# Autodesk Inventor assembly: Knee_MIR
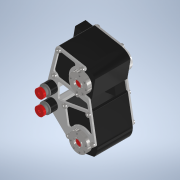
[picture p0: Inventor's stored thumbnail of the model, 180x180]
Saved by Autodesk Inventor 2020 (Build 240168000, 168)
## iProperties
Created: 2021-09-06
Part Number: Knee_MIR
Document SubType Name: Assembly
Designer: Masato Kubotera
Mass: 264.861 g
Surface Area: 473.637 cm^2
Volume: 130.531 cm^3
Density: 2.0291 g/cm^3
Author: Masato
## Documents named in this file (16)
- C:\Users\Masato\Desktop\OpenPlatform_ver3_0 - Ver4_1branch\LowerBody\Knee\Knee_MIR.iam
- C:\Users\Masato\Desktop\OpenPlatform_ver3_0 - Ver4_1branch\LowerBody\Knee\Knee_side_frame.ipt
- C:\Users\Masato\Desktop\OpenPlatform_ver3_0 - Ver4_1branch\Ready_Made\B3M11xx.ipt
- C:\Users\Masato\Desktop\OpenPlatform_ver3_0 - Ver4_1branch\Ready_Made\ClampHorn.ipt
- C:\Users\Masato\Desktop\OpenPlatform_ver3_0 - Ver4_1branch\Ready_Made\Screw\ClampHorn_Screw.ipt
- C:\Users\Masato\Desktop\OpenPlatform_ver3_0 - Ver4_1branch\Ready_Made\FreeHorn.ipt
- C:\Users\Masato\Desktop\OpenPlatform_ver3_0 - Ver4_1branch\Ready_Made\Screw\FreeHorn_Screw.ipt
- C:\Users\Masato\Desktop\OpenPlatform_ver3_0 - Ver4_1branch\Ready_Made\80F-0603.ipt
- C:\Users\Masato\Desktop\OpenPlatform_ver3_0 - Ver4_1branch\Ready_Made\Screw\M2_6-15.ipt
- C:\Users\Masato\Desktop\OpenPlatform_ver3_0 - Ver4_1branch\Ready_Made\Screw\M2_6-20.ipt
- C:\Users\Masato\Desktop\OpenPlatform_ver3_0 - Ver4_1branch\Ready_Made\UUW-0412-10BH.ipt
- C:\Users\Masato\Desktop\OpenPlatform_ver3_0 - Ver4_1branch\Ready_Made\CC-0612-15B.ipt
- C:\Users\Masato\Desktop\OpenPlatform_ver3_0 - Ver4_1branch\Ready_Made\CC-0612-50B.ipt
- C:\Users\Masato\Desktop\OpenPlatform_ver3_0 - Ver4_1branch\Ready_Made\SLSBF6-39_5-M4-N4.ipt
- C:\Users\Masato\Desktop\OpenPlatform_ver3_0 - Ver4_1branch\Ready_Made\DBTS4-11-6.ipt
- ClampHorn.ipt
## Components (50 placed, 14 different names)
1. Knee_side_frame:1 — フラッシュ:1, メイト:2, メイト:1, 挿入:6, 挿入:5, 挿入:8, 挿入:7, 挿入:3, 挿入:4, 挿入:1, 挿入:2, 挿入:9, 挿入:10, 挿入:12, 挿入:11, 挿入:13, 挿入:14, 挿入:15, 挿入:16, 角度:1, 挿入:33, 挿入:34, 挿入:37, 挿入:38
2. Knee_side_frame:2 — 挿入:22, 挿入:24, 挿入:21, 挿入:23, 挿入:20, 挿入:19, 挿入:18, 挿入:17, 挿入:26, 挿入:25, 挿入:28, 挿入:27, 挿入:31, 挿入:30, 挿入:32, 挿入:29, 挿入:35, 挿入:36, 挿入:39, 挿入:40
3. B3M11xx:1 — 挿入:20, 挿入:19, 挿入:3, 挿入:4, 挿入:18, 挿入:17, 挿入:1, 挿入:2, 挿入:61, 挿入:63, 挿入:59, 角度:3, 挿入:57
4. B3M11xx:2 — 挿入:6, 挿入:22, 挿入:24, 挿入:21, 挿入:23, 挿入:5, 挿入:8, 挿入:7, 挿入:62, 挿入:64, 挿入:60, 角度:4, 挿入:58
5. ClampHorn:1 — フラッシュ:2, 挿入:57, 角度:3
6. ClampHorn:2 — フラッシュ:3, 挿入:58, 角度:4
7. ClampHorn_Screw:1 — 挿入:59
8. ClampHorn_Screw:2 — 挿入:60
9. FreeHorn:1 — 挿入:61, フラッシュ:2
10. FreeHorn:2 — 挿入:62, フラッシュ:3
11. FreeHorn_Screw:1 — 挿入:63
12. FreeHorn_Screw:2 — 挿入:64
13. 80F-0603:1 — 挿入:49
14. 80F-0603:2 — 挿入:50
15. 80F-0603:3 — 挿入:51
16. 80F-0603:4 — 挿入:52
17. M2_6-15:1 — 挿入:9
18. M2_6-15:2 — 挿入:10
19. M2_6-15:3 — 挿入:11
20. M2_6-15:4 — 挿入:12
21. M2_6-15:5 — 挿入:13
22. M2_6-15:6 — 挿入:14
23. M2_6-15:7 — 挿入:15
24. M2_6-15:8 — 挿入:16
25. M2_6-20:1 — 挿入:25
26. M2_6-20:2 — 挿入:26
27. M2_6-20:3 — 挿入:27
28. M2_6-20:4 — 挿入:28
29. M2_6-20:5 — 挿入:29
30. M2_6-20:6 — 挿入:30
31. M2_6-20:7 — 挿入:31
32. M2_6-20:8 — 挿入:32
33. UUW-0412-10BH:1 — 挿入:53, 挿入:41, 挿入:37
34. UUW-0412-10BH:2 — 挿入:38, 挿入:54, 挿入:42
35. UUW-0412-10BH:3 — 挿入:55, 挿入:43, 挿入:39
36. UUW-0412-10BH:4 — 挿入:40, 挿入:56, 挿入:44
37. CC-0612-15B:1 — 挿入:45, 挿入:41
38. CC-0612-15B:2 — 挿入:46, 挿入:42
39. CC-0612-15B:3 — 挿入:47, 挿入:43
40. CC-0612-15B:4 — 挿入:48, 挿入:44
41. CC-0612-50B:1 — 挿入:49, 挿入:45
42. CC-0612-50B:2 — 挿入:50, 挿入:46
43. CC-0612-50B:3 — 挿入:51, 挿入:47
44. CC-0612-50B:4 — 挿入:52, 挿入:48
45. SLSBF6-39_5-M4-N4:1 — 角度:1, 挿入:33, 挿入:35, 角度:2
46. SLSBF6-39_5-M4-N4:2 — 挿入:36, 挿入:34, 角度:2
47. DBTS4-11-6:1 — 挿入:53
48. DBTS4-11-6:2 — 挿入:54
49. DBTS4-11-6:3 — 挿入:55
50. DBTS4-11-6:4 — 挿入:56
## Relationships (73: Insert 64, Angle 4, Flush 3, Mate 2)
- フラッシュ:1 [Flush]: Knee_side_frame:1
- メイト:2 [Mate] (19.75 mm): Knee_side_frame:1
- メイト:1 [Mate]: Knee_side_frame:1
- 挿入:6 [Insert]: Knee_side_frame:1 ↔ B3M11xx:2
- 挿入:22 [Insert]: Knee_side_frame:2 ↔ B3M11xx:2
- 挿入:24 [Insert]: Knee_side_frame:2 ↔ B3M11xx:2
- 挿入:21 [Insert]: Knee_side_frame:2 ↔ B3M11xx:2
- 挿入:23 [Insert]: Knee_side_frame:2 ↔ B3M11xx:2
- 挿入:5 [Insert]: Knee_side_frame:1 ↔ B3M11xx:2
- 挿入:8 [Insert]: Knee_side_frame:1 ↔ B3M11xx:2
- 挿入:7 [Insert]: Knee_side_frame:1 ↔ B3M11xx:2
- 挿入:20 [Insert]: Knee_side_frame:2 ↔ B3M11xx:1
- 挿入:19 [Insert]: Knee_side_frame:2 ↔ B3M11xx:1
- 挿入:3 [Insert]: Knee_side_frame:1 ↔ B3M11xx:1
- 挿入:4 [Insert]: Knee_side_frame:1 ↔ B3M11xx:1
- 挿入:18 [Insert]: Knee_side_frame:2 ↔ B3M11xx:1
- 挿入:17 [Insert]: Knee_side_frame:2 ↔ B3M11xx:1
- 挿入:1 [Insert]: Knee_side_frame:1 ↔ B3M11xx:1
- 挿入:2 [Insert]: Knee_side_frame:1 ↔ B3M11xx:1
- 挿入:62 [Insert]: B3M11xx:2 ↔ FreeHorn:2
- 挿入:61 [Insert]: B3M11xx:1 ↔ FreeHorn:1
- 挿入:9 [Insert]: Knee_side_frame:1 ↔ M2_6-15:1
- 挿入:10 [Insert]: Knee_side_frame:1 ↔ M2_6-15:2
- 挿入:12 [Insert]: Knee_side_frame:1 ↔ M2_6-15:4
- 挿入:11 [Insert]: Knee_side_frame:1 ↔ M2_6-15:3
- 挿入:13 [Insert]: Knee_side_frame:1 ↔ M2_6-15:5
- 挿入:14 [Insert]: Knee_side_frame:1 ↔ M2_6-15:6
- 挿入:15 [Insert]: Knee_side_frame:1 ↔ M2_6-15:7
- 挿入:16 [Insert]: Knee_side_frame:1 ↔ M2_6-15:8
- 挿入:26 [Insert]: Knee_side_frame:2 ↔ M2_6-20:2
- 挿入:25 [Insert]: Knee_side_frame:2 ↔ M2_6-20:1
- 挿入:28 [Insert]: Knee_side_frame:2 ↔ M2_6-20:4
- 挿入:27 [Insert]: Knee_side_frame:2 ↔ M2_6-20:3
- 挿入:31 [Insert]: Knee_side_frame:2 ↔ M2_6-20:7
- 挿入:30 [Insert]: Knee_side_frame:2 ↔ M2_6-20:6
- 挿入:32 [Insert]: Knee_side_frame:2 ↔ M2_6-20:8
- 挿入:29 [Insert]: Knee_side_frame:2 ↔ M2_6-20:5
- 挿入:50 [Insert]: 80F-0603:2 ↔ CC-0612-50B:2
- 挿入:46 [Insert]: CC-0612-15B:2 ↔ CC-0612-50B:2
- 挿入:49 [Insert]: 80F-0603:1 ↔ CC-0612-50B:1
- 挿入:45 [Insert]: CC-0612-15B:1 ↔ CC-0612-50B:1
- 挿入:51 [Insert]: 80F-0603:3 ↔ CC-0612-50B:3
- 挿入:47 [Insert]: CC-0612-15B:3 ↔ CC-0612-50B:3
- 挿入:52 [Insert]: 80F-0603:4 ↔ CC-0612-50B:4
- 挿入:48 [Insert]: CC-0612-15B:4 ↔ CC-0612-50B:4
- 挿入:64 [Insert]: B3M11xx:2 ↔ FreeHorn_Screw:2
- 挿入:63 [Insert]: B3M11xx:1 ↔ FreeHorn_Screw:1
- 角度:1 [Angle] (0 deg): Knee_side_frame:1 ↔ SLSBF6-39_5-M4-N4:1
- 挿入:33 [Insert]: Knee_side_frame:1 ↔ SLSBF6-39_5-M4-N4:1
- 挿入:35 [Insert]: Knee_side_frame:2 ↔ SLSBF6-39_5-M4-N4:1
- 挿入:36 [Insert]: Knee_side_frame:2 ↔ SLSBF6-39_5-M4-N4:2
- 挿入:34 [Insert]: Knee_side_frame:1 ↔ SLSBF6-39_5-M4-N4:2
- 角度:2 [Angle] (0 deg): SLSBF6-39_5-M4-N4:1 ↔ SLSBF6-39_5-M4-N4:2
- 挿入:53 [Insert]: UUW-0412-10BH:1 ↔ DBTS4-11-6:1
- 挿入:41 [Insert]: UUW-0412-10BH:1 ↔ CC-0612-15B:1
- 挿入:37 [Insert]: Knee_side_frame:1 ↔ UUW-0412-10BH:1
- 挿入:38 [Insert]: Knee_side_frame:1 ↔ UUW-0412-10BH:2
- 挿入:54 [Insert]: UUW-0412-10BH:2 ↔ DBTS4-11-6:2
- 挿入:42 [Insert]: UUW-0412-10BH:2 ↔ CC-0612-15B:2
- 挿入:55 [Insert]: UUW-0412-10BH:3 ↔ DBTS4-11-6:3
- 挿入:43 [Insert]: UUW-0412-10BH:3 ↔ CC-0612-15B:3
- 挿入:39 [Insert]: Knee_side_frame:2 ↔ UUW-0412-10BH:3
- 挿入:40 [Insert]: Knee_side_frame:2 ↔ UUW-0412-10BH:4
- 挿入:56 [Insert]: UUW-0412-10BH:4 ↔ DBTS4-11-6:4
- 挿入:44 [Insert]: UUW-0412-10BH:4 ↔ CC-0612-15B:4
- 挿入:59 [Insert]: B3M11xx:1 ↔ ClampHorn_Screw:1
- 挿入:60 [Insert]: B3M11xx:2 ↔ ClampHorn_Screw:2
- フラッシュ:3 [Flush]: ClampHorn:2 ↔ FreeHorn:2
- 角度:4 [Angle] (0 deg): B3M11xx:2 ↔ ClampHorn:2
- 挿入:58 [Insert]: B3M11xx:2 ↔ ClampHorn:2
- フラッシュ:2 [Flush]: ClampHorn:1 ↔ FreeHorn:1
- 角度:3 [Angle] (0 deg): B3M11xx:1 ↔ ClampHorn:1
- 挿入:57 [Insert]: B3M11xx:1 ↔ ClampHorn:1
